# Autodesk Inventor assembly: Robot Dog
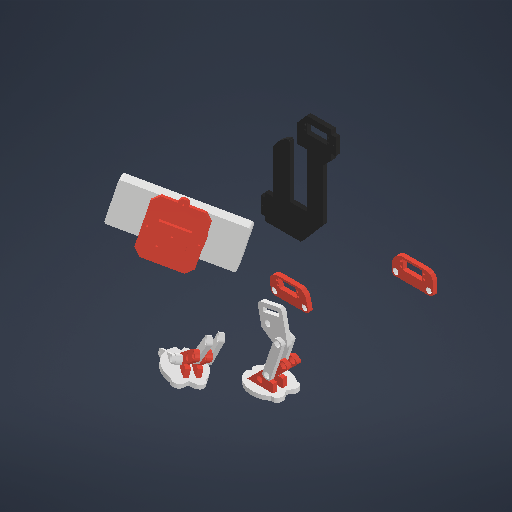
[picture p0: Inventor's stored thumbnail of the model, 512x512]
Saved by Autodesk Inventor 2026.2 (Build 302298010, 298A)
## iProperties
Created: 2026-07-03
Part Number: Robot Dog
Document SubType Name: Assembly
Designer: Martina
Author: Martina
## Documents named in this file (12)
- D:\Semester 4\Praktikum Robotika\3d inventor\Robot Dog.iam
- D:\Semester 4\Praktikum Robotika\Project Robotika\Project Robotika\telapak kaki_MIR.ipt
- D:\Semester 4\Praktikum Robotika\Project Robotika\Project Robotika\Body Lengan Kaki\Component2_MIR.ipt
- D:\Semester 4\Praktikum Robotika\Project Robotika\YouCanBuildDog-main\YouCanBuildDog-main\CAD\dog02_large\dog02_large\Buat Ulang\Uleg01_MIR.ipt
- D:\Semester 4\Praktikum Robotika\Project Robotika\YouCanBuildDog-main\YouCanBuildDog-main\CAD\dog02_large\dog02_large\Buat Ulang\Spacer6_MIR.ipt
- D:\Semester 4\Praktikum Robotika\Project Robotika\YouCanBuildDog-main\YouCanBuildDog-main\CAD\dog02_large\dog02_large\Buat Ulang\LegLver_MIR.ipt
- D:\Semester 4\Praktikum Robotika\Project Robotika\YouCanBuildDog-main\YouCanBuildDog-main\CAD\dog02_large\dog02_large\Buat Ulang\Hip.ipt
- D:\Semester 4\Praktikum Robotika\Project Robotika\Project Robotika\KEPALA.ipt
- D:\Semester 4\Praktikum Robotika\Project Robotika\Project Robotika\Leher Robot.ipt
- D:\Semester 4\Praktikum Robotika\Project Robotika\Project Robotika\Atas Slider.ipt
- D:\Semester 4\Praktikum Robotika\Project Robotika\Project Robotika\Body Slider Hitam\Component4.ipt
- D:\Semester 4\Praktikum Robotika\Project Robotika\Project Robotika\Body Kaki Servo\Component2_MIR.ipt
## Components (21 placed, 10 different names)
1. telapak kaki_MIR:2 — Mate:1, Mate:2, Mate:3, Mate:4, Mate:5, Mate:6
2. Component2_MIR:2 — Mate:3, Mate:4, Mate:6, Rotational:3, Rotational:5
3. Component2_MIR:4 — Mate:1, Mate:2, Mate:5, Rotational:6
4. telapak kaki_MIR:6
5. Component2_MIR:10 — Rotational:1, Rotational:7
6. Component2_MIR:11 — Rotational:8
7. Uleg01_MIR:1 — Rotational:2
8. Uleg01_MIR:3 — Rotational:4
9. Spacer6_MIR:1 — Rotational:1, Rotational:2
10. Spacer6_MIR:2 — Rotational:3, Rotational:4
11. LegLver_MIR:1 — Rotational:5, Mate:38
12. LegLver_MIR:2 — Rotational:6, Mate:39
13. Hip:2 — Mate:38, Mate:39
14. KEPALA:1 — Mate:32, Mate:33, Mate:34
15. Leher Robot:1 — Mate:32, Mate:33, Mate:34, Mate:35, Mate:36, Mate:37
16. Atas Slider:1 — Mate:35, Mate:36, Mate:37
17. LegLver_MIR:3 — Rotational:7
18. LegLver_MIR:4 — Rotational:8
19. Component4:1
20. Component2_MIR:12
21. Component2_MIR:13
## Relationships (30: Mate 22, RevoluteJoint 8)
- Mate:1: telapak kaki_MIR:2 ↔ Component2_MIR:4
- Mate:2: telapak kaki_MIR:2 ↔ Component2_MIR:4
- Mate:3: telapak kaki_MIR:2 ↔ Component2_MIR:2
- Mate:4: telapak kaki_MIR:2 ↔ Component2_MIR:2
- Mate:5: telapak kaki_MIR:2 ↔ Component2_MIR:4
- Mate:6: telapak kaki_MIR:2 ↔ Component2_MIR:2
- [Mate]: telapak kaki_MIR:6 ↔ Component2_MIR:10
- [Mate]: telapak kaki_MIR:6 ↔ Component2_MIR:10
- [Mate]: telapak kaki_MIR:6 ↔ Component2_MIR:10
- [Mate]: telapak kaki_MIR:6 ↔ Component2_MIR:10
- [Mate]: telapak kaki_MIR:6 ↔ Component2_MIR:11
- [Mate]: telapak kaki_MIR:6 ↔ Component2_MIR:11
- [Mate]: telapak kaki_MIR:6 ↔ Component2_MIR:11
- [Mate]: telapak kaki_MIR:6 ↔ Component2_MIR:11
- Rotational:1 [RevoluteJoint]: Component2_MIR:10 ↔ Spacer6_MIR:1
- Rotational:2 [RevoluteJoint]: Uleg01_MIR:1 ↔ Spacer6_MIR:1
- Rotational:3 [RevoluteJoint]: Component2_MIR:2 ↔ Spacer6_MIR:2
- Rotational:4 [RevoluteJoint]: Uleg01_MIR:3 ↔ Spacer6_MIR:2
- Rotational:5 [RevoluteJoint] (1.27 mm): Component2_MIR:2 ↔ LegLver_MIR:1
- Rotational:6 [RevoluteJoint] (1.524 mm): Component2_MIR:4 ↔ LegLver_MIR:2
- Mate:32: KEPALA:1 ↔ Leher Robot:1
- Mate:33: KEPALA:1 ↔ Leher Robot:1
- Mate:34: KEPALA:1 ↔ Leher Robot:1
- Mate:35: Leher Robot:1 ↔ Atas Slider:1
- Mate:36: Leher Robot:1 ↔ Atas Slider:1
- Mate:37: Leher Robot:1 ↔ Atas Slider:1
- Rotational:7 [RevoluteJoint] (1.016 mm): Component2_MIR:10 ↔ LegLver_MIR:3
- Rotational:8 [RevoluteJoint] (1.016 mm): Component2_MIR:11 ↔ LegLver_MIR:4
- Mate:38 (1 mm): LegLver_MIR:1 ↔ Hip:2
- Mate:39: LegLver_MIR:2 ↔ Hip:2
## Named parameters: d20_d12 = 0 mm, d21_d13 = 0 mm, d22_d14 = 0 mm, d23_d15 = 0 mm, d24_d16 = 0 mm, d25_d17 = 0 mm, d26_d18 = 0 mm, d27_d19 = 0 mm
